# Autodesk Inventor assembly: Desk Assembly
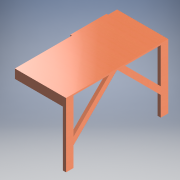
[picture p0: Inventor's stored thumbnail of the model, 180x180]
Saved by Autodesk Inventor 2018 (Build 220112000, 112)
## iProperties
Created: 2016-08-30
Part Number: Desk Assembly
Document SubType Name: Assembly
Designer: jjsch
Mass: 38826.1 g
Surface Area: 62997.1 cm^2
Volume: 68085.2 cm^3
Density: 0.570257 g/cm^3
Author: jjsch
## Documents named in this file (15)
- G:\Justin_C\jjsch\Documents\Engineering\Desk V2.1\Addon Section.iam
- G:\Justin_C\jjsch\Documents\Engineering\Desk V2.1\Joist, Side.ipt
- G:\Justin_C\jjsch\Documents\Engineering\Desk V2.1\Back Angle Piece.ipt
- G:\Justin_C\jjsch\Documents\Engineering\Desk V2.1\Top Continuation Bar.ipt
- G:\Justin_C\jjsch\Documents\Engineering\Desk V2.1\LTabletop.ipt
- G:\Justin_C\jjsch\Documents\Engineering\Desk V2.1\LongColumn.ipt
- G:\Justin_C\jjsch\Documents\Engineering\Desk V2.1\LSideBar.ipt
- G:\Justin_C\jjsch\Documents\Engineering\Desk V2.1\AesteticTriangle.ipt
- G:\Justin_C\jjsch\Documents\Engineering\Desk V2.1\LBackAnglePiece.ipt
- G:\Justin_C\jjsch\Documents\Engineering\Desk V2.1\Addon Section\AIP\FEA\c9kno9v34.fins
- G:\Justin_C\jjsch\Documents\Engineering\Desk V2.1\Addon Section\AIP\FEA\c9kno9v34.fsat
- G:\Justin_C\jjsch\Documents\Engineering\Desk V2.1\Addon Section\AIP\FEA\c9kno9v34.ftes
- G:\Justin_C\jjsch\Documents\Engineering\Desk V2.1\Addon Section\AIP\FEA\c9kno9v34.fwiz
- G:\Justin_C\jjsch\Documents\Engineering\Desk V2.1\Addon Section\AIP\FEA\c9kno9v4w.fmsh
- G:\Justin_C\jjsch\Documents\Engineering\Desk V2.1\Addon Section\AIP\FEA\c9kno9v5s.fres
## Components (10 placed, 8 different names)
1. Joist, Side:1
2. Top Continuation Bar:1 — Flush:18
3. LTabletop:1 — Flush:18, Flush:20, Mate:23, Mate:24, Flush:21, Flush:22, Mate:26, Flush:26, Flush:29, Flush:30, Mate:31, Flush:33, Mate:32, Mate:33
4. LongColumn:1 — Mate:24, Flush:21, Flush:22, Mate:35, Flush:35
5. LongColumn:2 — Flush:20, Mate:23, Flush:26, Mate:34, Flush:34
6. Back Angle Piece:3 — Mate:26
7. LSideBar:1 — Flush:29, Flush:30, Mate:31, Flush:31, Flush:32
8. AesteticTriangle:1 — Flush:31, Flush:32, Flush:33
9. LBackAnglePiece:1 — Mate:33, Mate:35, Flush:35
10. LBackAnglePiece:2 — Mate:32, Mate:34, Flush:34
## Relationships (20: Flush 12, Mate 8)
- Flush:18: Top Continuation Bar:1 ↔ LTabletop:1
- Flush:20: LTabletop:1 ↔ LongColumn:2
- Mate:23: LTabletop:1 ↔ LongColumn:2
- Mate:24: LTabletop:1 ↔ LongColumn:1
- Flush:21: LTabletop:1 ↔ LongColumn:1
- Flush:22: LTabletop:1 ↔ LongColumn:1
- Mate:26: LTabletop:1 ↔ Back Angle Piece:3
- Flush:26: LTabletop:1 ↔ LongColumn:2
- Flush:29: LTabletop:1 ↔ LSideBar:1
- Flush:30: LTabletop:1 ↔ LSideBar:1
- Mate:31: LTabletop:1 ↔ LSideBar:1
- Flush:31: LSideBar:1 ↔ AesteticTriangle:1
- Flush:32: LSideBar:1 ↔ AesteticTriangle:1
- Flush:33: LTabletop:1 ↔ AesteticTriangle:1
- Mate:32: LTabletop:1 ↔ LBackAnglePiece:2
- Mate:33: LTabletop:1 ↔ LBackAnglePiece:1
- Mate:34: LongColumn:2 ↔ LBackAnglePiece:2
- Mate:35: LongColumn:1 ↔ LBackAnglePiece:1
- Flush:34: LongColumn:2 ↔ LBackAnglePiece:2
- Flush:35: LongColumn:1 ↔ LBackAnglePiece:1
## Named parameters: sa_0 = 133447
note: some values were not read from the file. Shown as the stored number, unit unknown: "sa_0".
